# Autodesk Inventor assembly: Motor Assembly
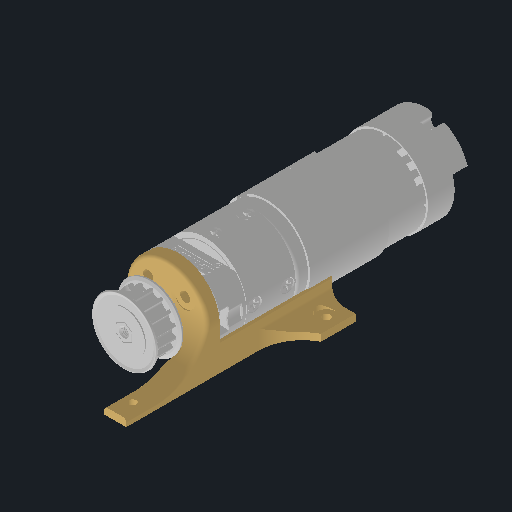
[picture p0: Inventor's stored thumbnail of the model, 512x512]
Saved by Autodesk Inventor 2022 (Build 260153000, 153)
## iProperties
Created: 2021-11-02
Part Number: Motor Assembly
Document SubType Name: Assembly
Designer: divid
Author: divid
## Documents named in this file (4)
- C:\Users\divid\Documents\GitHub\ComputerAidedDesign\2021-22\FTC\#13822 Robovikes\Drivetrain\Motor Assemblies\Motor Assembly (Left).iam
- C:\Users\divid\Documents\GitHub\ComputerAidedDesign\2021-22\FTC\#13822 Robovikes\Drivetrain\Motor Assemblies\Yellow Jacket Motor\5203 Series Yellow Jacket Planetary Gear Motor (1620 RPM).iam
- C:\Users\divid\Documents\GitHub\ComputerAidedDesign\2021-22\FTC\#13822 Robovikes\Drivetrain\Timing Belt Pulley (8mm REX Bore, 16 Tooth)\3414 Series 5mm HTD Pitch Set Screw Pinion Timing Belt Pulley (8mm REX Bore, 16 Tooth).iam
- C:\Users\divid\Documents\GitHub\ComputerAidedDesign\2021-22\FTC\#13822 Robovikes\Drivetrain\Motor Assemblies\Custom GoBilda Yellow Jacket Motor Mount (Back).ipt
## Components (3 placed, 3 different names)
1. 5203 Series Yellow Jacket Planetary Gear Motor (1620 RPM):1 [sub-assembly] — Mate:3
2. Custom GoBilda Yellow Jacket Motor Mount (Back):2 — Mate:3
3. 3414 Series 5mm HTD Pitch Set Screw Pinion Timing Belt Pulley (8mm REX Bore, 16 Tooth):1 [sub-assembly]
## Relationships (6: Mate 5, Flush 1)
- [Mate]: 5203 Series Yellow Jacket Planetary Gear Motor (1620 RPM):1 ↔ Custom GoBilda Yellow Jacket Motor Mount (Back):2
- [Mate]: 5203 Series Yellow Jacket Planetary Gear Motor (1620 RPM):1 ↔ Custom GoBilda Yellow Jacket Motor Mount (Back):2
- Mate:3: 5203 Series Yellow Jacket Planetary Gear Motor (1620 RPM):1 ↔ Custom GoBilda Yellow Jacket Motor Mount (Back):2
- [Mate]: 5203 Series Yellow Jacket Planetary Gear Motor (1620 RPM):1 ↔ 3414 Series 5mm HTD Pitch Set Screw Pinion Timing Belt Pulley (8mm REX Bore, 16 Tooth):1
- [Mate]: 5203 Series Yellow Jacket Planetary Gear Motor (1620 RPM):1 ↔ 3414 Series 5mm HTD Pitch Set Screw Pinion Timing Belt Pulley (8mm REX Bore, 16 Tooth):1
- [Flush]: 5203 Series Yellow Jacket Planetary Gear Motor (1620 RPM):1 ↔ 3414 Series 5mm HTD Pitch Set Screw Pinion Timing Belt Pulley (8mm REX Bore, 16 Tooth):1
